# Autodesk Inventor assembly: crio
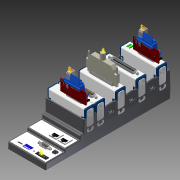
[picture p0: Inventor's stored thumbnail of the model, 180x180]
Saved by Autodesk Inventor 2011 (Build 150239000, 239)
## iProperties
Created: 2010-02-10
Part Number: crio
Document SubType Name: Assembly
Designer: a
Author: a
## Documents named in this file (9)
- R:\2012\Inventor\vkop\All-Control-System\CRIO_ASMB.iam
- R:\2012\Inventor\vkop\All-Control-System\Control System_NI_NI-cRIO-FRC.ipt
- R:\2012\Inventor\vkop\All-Control-System\Control System_Diversified_Systems_A003265.ipt
- R:\2012\Inventor\vkop\All-Control-System\Control System_NI_9201.ipt
- R:\2012\Inventor\vkop\All-Control-System\Control System_NI_9403.ipt
- R:\2012\Inventor\vkop\All-Control-System\Control System_NI_9472.ipt
- \\Lmss\students\Robotics\Inventor\I_Team\elect\ethernet connector red.ipt
- \\Lmss\students\Robotics\Inventor\I_Team\elect\ethernet connector.ipt
- R:\2012\Inventor\vkop\All-Electrical\37 pin connector.ipt
## Components (11 placed, 8 different names)
1. Control System_NI_NI-cRIO-FRC:1 — Mate:1, Mate:2, Mate:3, Mate:4, Mate:5, Mate:6, Mate:7, Mate:8, Mate:9, Mate:10, Mate:11, Mate:14, Mate:15, Mate:16, Mate:17, Mate:18, Mate:19
2. Control System_Diversified_Systems_A003265:1 — Flush:5, Mate:12, Mate:13
3. Control System_NI_9201:1 — Mate:1, Mate:2, Mate:5, Flush:1, Flush:2, Flush:3, Flush:4, Flush:5, Mate:12, Mate:13
4. Control System_NI_9201:2 — Mate:3, Mate:4, Flush:1
5. Control System_NI_9403:1 — Mate:6, Mate:7, Flush:2, Mate:24, Mate:25
6. Control System_NI_9403:2 — Mate:8, Mate:9, Flush:3, Mate:23
7. Control System_NI_9472:1 — Mate:10, Mate:11, Flush:4, Mate:20, Mate:21, Mate:22
8. ethernet connector red:1 — Mate:14, Mate:15, Mate:16
9. ethernet connector:1 — Mate:17, Mate:18, Mate:19
10. Control System_Diversified_Systems_A003265:2 — Mate:20, Mate:21, Mate:22
11. 37 pin connector:1 — Mate:23, Mate:24, Mate:25
## Relationships (30: Mate 25, Flush 5)
- Mate:1: Control System_NI_NI-cRIO-FRC:1 ↔ Control System_NI_9201:1
- Mate:2: Control System_NI_NI-cRIO-FRC:1 ↔ Control System_NI_9201:1
- Mate:3: Control System_NI_NI-cRIO-FRC:1 ↔ Control System_NI_9201:2
- Mate:4: Control System_NI_NI-cRIO-FRC:1 ↔ Control System_NI_9201:2
- Mate:5: Control System_NI_NI-cRIO-FRC:1 ↔ Control System_NI_9201:1
- Flush:1: Control System_NI_9201:1 ↔ Control System_NI_9201:2
- Mate:6: Control System_NI_NI-cRIO-FRC:1 ↔ Control System_NI_9403:1
- Mate:7: Control System_NI_NI-cRIO-FRC:1 ↔ Control System_NI_9403:1
- Flush:2: Control System_NI_9201:1 ↔ Control System_NI_9403:1
- Mate:8: Control System_NI_NI-cRIO-FRC:1 ↔ Control System_NI_9403:2
- Mate:9: Control System_NI_NI-cRIO-FRC:1 ↔ Control System_NI_9403:2
- Flush:3: Control System_NI_9201:1 ↔ Control System_NI_9403:2
- Mate:10: Control System_NI_NI-cRIO-FRC:1 ↔ Control System_NI_9472:1
- Mate:11: Control System_NI_NI-cRIO-FRC:1 ↔ Control System_NI_9472:1
- Flush:4: Control System_NI_9201:1 ↔ Control System_NI_9472:1
- Flush:5: Control System_Diversified_Systems_A003265:1 ↔ Control System_NI_9201:1
- Mate:12: Control System_Diversified_Systems_A003265:1 ↔ Control System_NI_9201:1
- Mate:13: Control System_Diversified_Systems_A003265:1 ↔ Control System_NI_9201:1
- Mate:14: Control System_NI_NI-cRIO-FRC:1 ↔ ethernet connector red:1
- Mate:15: Control System_NI_NI-cRIO-FRC:1 ↔ ethernet connector red:1
- Mate:16: Control System_NI_NI-cRIO-FRC:1 ↔ ethernet connector red:1
- Mate:17: Control System_NI_NI-cRIO-FRC:1 ↔ ethernet connector:1
- Mate:18: Control System_NI_NI-cRIO-FRC:1 ↔ ethernet connector:1
- Mate:19: Control System_NI_NI-cRIO-FRC:1 ↔ ethernet connector:1
- Mate:20: Control System_NI_9472:1 ↔ Control System_Diversified_Systems_A003265:2
- Mate:21: Control System_NI_9472:1 ↔ Control System_Diversified_Systems_A003265:2
- Mate:22: Control System_NI_9472:1 ↔ Control System_Diversified_Systems_A003265:2
- Mate:23: Control System_NI_9403:2 ↔ 37 pin connector:1
- Mate:24: Control System_NI_9403:1 ↔ 37 pin connector:1
- Mate:25: Control System_NI_9403:1 ↔ 37 pin connector:1
